# Autodesk Inventor assembly: Assembly1
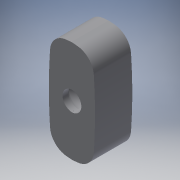
[picture p0: Inventor's stored thumbnail of the model, 180x180]
Saved by Autodesk Inventor 2017 (Build 210142000, 142)
## iProperties
Created: 2019-06-26
Part Number: Assembly1
Document SubType Name: Assembly
Designer: Ole Simmering
Author: Ole Simmering
## Documents named in this file (4)
- C:\Users\Ole Simmering\Documents\GitHub\3D_modeling\Kopfhörer Ersatzteil\Assembly1.iam
- C:\Users\Ole Simmering\Documents\GitHub\3D_modeling\Kopfhörer Ersatzteil\Part1.ipt
- C:\Users\Ole Simmering\Documents\GitHub\3D_modeling\Kopfhörer Ersatzteil\Part2.ipt
- C:\Users\Ole Simmering\Documents\Inventor\Content Center Files\R2017\en-US\AS 1427(04)\AS 1427 - M2 x 8(5) I.ipt
## Components (4 placed, 3 different names)
1. Part1:1 — Angle:1, Mate:1, Mate:2, Insert:1
2. Part2:1 — Angle:1, Mate:1, Mate:2, Insert:1, Insert:2, Insert:3
3. AS 1427 H - Metric M2 x 8:1 — Insert:3
4. AS 1427 H - Metric M2 x 8:2 — Insert:2
## Relationships (6: Insert 3, Mate 2, Angle 1)
- Angle:1 (0 deg): Part1:1 ↔ Part2:1
- Mate:1: Part1:1 ↔ Part2:1
- Mate:2: Part1:1 ↔ Part2:1
- Insert:1: Part1:1 ↔ Part2:1
- Insert:2 (1 mm): Part2:1 ↔ AS 1427 H - Metric M2 x 8:2
- Insert:3 (1 mm): Part2:1 ↔ AS 1427 H - Metric M2 x 8:1
